# Autodesk Inventor assembly: манипулятор 2
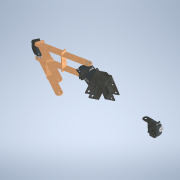
[picture p0: Inventor's stored thumbnail of the model, 180x180]
Saved by Autodesk Inventor 2020.1 (Build 241239000, 239)
## iProperties
Created: 2021-08-18
Part Number: манипулятор 2
Document SubType Name: Assembly
Designer: User
Author: User
## Documents named in this file (11)
- D:\GitHub\avatar-kvantoriada\3D\манипулятор 2.iam
- D:\GitHub\avatar-kvantoriada\3D\основа.ipt
- D:\GitHub\avatar-kvantoriada\3D\основа_ЗЕРКАЛО.ipt
- D:\GitHub\avatar-kvantoriada\3D\сборка серва 90.iam
- D:\GitHub\avatar-kvantoriada\3D\сборка серва 45_ЗЕРКАЛО.iam
- D:\GitHub\avatar-kvantoriada\3D\Сборка1.iam
- D:\GitHub\avatar-kvantoriada\3D\подшипник.iam
- D:\GitHub\avatar-kvantoriada\3D\сборка серва 90_ЗЕРКАЛО_ЗЕРКАЛО.iam
- D:\GitHub\avatar-kvantoriada\3D\Сборка2.iam
- D:\GitHub\avatar-kvantoriada\3D\уголок.ipt
- C:\Users\User\Documents\Inventor\Content Center Files\R2020\ru-RU\AS 1427(08)\AS 1427 - M3 x 8(6) I.ipt
## Components (24 placed, 10 different names)
1. основа:2 — С поворотом:1
2. основа_ЗЕРКАЛО:1 — С поворотом:1, С поворотом:2
3. сборка серва 90:2 [sub-assembly] — С поворотом:2, С поворотом:3
4. сборка серва 45_ЗЕРКАЛО:1 [sub-assembly] — С поворотом:3, С поворотом:4, Жесткий:1
5. Сборка1:1 [sub-assembly] — С поворотом:4, С поворотом:5, Жесткий:10, Жесткий:11, Жесткий:12, Жесткий:13, Жесткий:14, Жесткий:15, Жесткий:16, Жесткий:17
6. подшипник:1 [sub-assembly] — Жесткий:1
7. сборка серва 90_ЗЕРКАЛО_ЗЕРКАЛО:1 [sub-assembly] — С поворотом:5, С поворотом:6, Жесткий:4
8. Сборка2:1 [sub-assembly] — Жесткий:2, Жесткий:6, Жесткий:7, Жесткий:8, Жесткий:9
9. уголок:1 — С поворотом:6, Жесткий:2
10. сборка серва 90:3 [sub-assembly] — Жесткий:3
11. уголок:2 — Жесткий:3
12. подшипник:2 [sub-assembly] — Жесткий:4
13. AS 1427 Z - метрическая M3 x 8:7 — Жесткий:7
14. AS 1427 Z - метрическая M3 x 8:9 — Жесткий:12
15. AS 1427 Z - метрическая M3 x 8:10 — Жесткий:9
16. AS 1427 Z - метрическая M3 x 8:11 — Жесткий:8
17. AS 1427 Z - метрическая M3 x 8:12 — Жесткий:6
18. AS 1427 Z - метрическая M3 x 8:13 — Жесткий:13
19. AS 1427 Z - метрическая M3 x 8:14 — Жесткий:10
20. AS 1427 Z - метрическая M3 x 8:15 — Жесткий:11
21. AS 1427 Z - метрическая M3 x 8:16 — Жесткий:14
22. AS 1427 Z - метрическая M3 x 8:17 — Жесткий:16
23. AS 1427 Z - метрическая M3 x 8:20 — Жесткий:17
24. AS 1427 Z - метрическая M3 x 8:21 — Жесткий:15
## Relationships (22: WeldJoint 16, RevoluteJoint 6)
- С поворотом:1 [RevoluteJoint]: основа:2 ↔ основа_ЗЕРКАЛО:1
- С поворотом:2 [RevoluteJoint]: основа_ЗЕРКАЛО:1 ↔ сборка серва 90:2
- С поворотом:3 [RevoluteJoint]: сборка серва 90:2 ↔ сборка серва 45_ЗЕРКАЛО:1
- С поворотом:4 [RevoluteJoint]: сборка серва 45_ЗЕРКАЛО:1 ↔ Сборка1:1
- Жесткий:1 [WeldJoint]: сборка серва 45_ЗЕРКАЛО:1 ↔ подшипник:1
- С поворотом:5 [RevoluteJoint]: Сборка1:1 ↔ сборка серва 90_ЗЕРКАЛО_ЗЕРКАЛО:1
- С поворотом:6 [RevoluteJoint]: сборка серва 90_ЗЕРКАЛО_ЗЕРКАЛО:1 ↔ уголок:1
- Жесткий:2 [WeldJoint]: Сборка2:1 ↔ уголок:1
- Жесткий:3 [WeldJoint]: сборка серва 90:3 ↔ уголок:2
- Жесткий:4 [WeldJoint]: сборка серва 90_ЗЕРКАЛО_ЗЕРКАЛО:1 ↔ подшипник:2
- Жесткий:6 [WeldJoint]: Сборка2:1 ↔ AS 1427 Z - метрическая M3 x 8:12
- Жесткий:7 [WeldJoint]: Сборка2:1 ↔ AS 1427 Z - метрическая M3 x 8:7
- Жесткий:8 [WeldJoint]: Сборка2:1 ↔ AS 1427 Z - метрическая M3 x 8:11
- Жесткий:9 [WeldJoint]: Сборка2:1 ↔ AS 1427 Z - метрическая M3 x 8:10
- Жесткий:10 [WeldJoint]: Сборка1:1 ↔ AS 1427 Z - метрическая M3 x 8:14
- Жесткий:11 [WeldJoint]: Сборка1:1 ↔ AS 1427 Z - метрическая M3 x 8:15
- Жесткий:12 [WeldJoint]: Сборка1:1 ↔ AS 1427 Z - метрическая M3 x 8:9
- Жесткий:13 [WeldJoint]: Сборка1:1 ↔ AS 1427 Z - метрическая M3 x 8:13
- Жесткий:14 [WeldJoint]: Сборка1:1 ↔ AS 1427 Z - метрическая M3 x 8:16
- Жесткий:15 [WeldJoint]: Сборка1:1 ↔ AS 1427 Z - метрическая M3 x 8:21
- Жесткий:16 [WeldJoint]: Сборка1:1 ↔ AS 1427 Z - метрическая M3 x 8:17
- Жесткий:17 [WeldJoint]: Сборка1:1 ↔ AS 1427 Z - метрическая M3 x 8:20
